(part 1 of 4)
# Autodesk Inventor assembly: 000 Ensamblaje hw_LM - BASIC
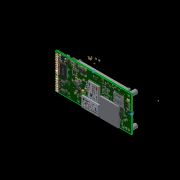
[picture p0: Inventor's stored thumbnail of the model, 180x180]
Saved by Autodesk Inventor 2018.3 (Build 223284000, 284)
## iProperties
Created: 2025-09-15
Part Number: 000 Ensamblaje hw_LM - BASIC
Document SubType Name: Assembly
Designer: mbs18
Mass: 915.711 g
Surface Area: 945.94 cm^2
Volume: 71.5532 cm^3
Density: 12.7976 g/cm^3
Author: mbs18
## Documents named in this file (64)
- C:\Users\mbs18.Embention\Git\LM\items\3d_LM\hw_LM\3d\000 Ensamblaje hw_LM - BASIC.iam
- C:\Users\mbs18.Embention\Git\LM\items\3d_LM\hw_LM\3d\hw_LM - PCB.ipt
- C:\Users\mbs18.Embention\Git\LM\items\_accesories\Componentes PCB\Conectores\3d_Molex\3d\47219-2001\47219-2001.ipt
- C:\Users\mbs18.Embention\Git\LM\items\_accesories\Componentes PCB\Magnetometro\3d_PNI Corp\3d\RM3100\Sen-XY-f.ipt
- C:\Users\mbs18.Embention\Git\LM\items\_accesories\Componentes PCB\Magnetometro\3d_PNI Corp\3d\RM3100\Sen-Z-f.ipt
- C:\Users\mbs18.Embention\Git\LM\items\_accesories\Componentes PCB\Conectores\3d_Samtec\3d\CLP-104-02-F-D-BE-TR.ipt
- C:\Users\mbs18.Embention\Git\LM\items\_accesories\Componentes PCB\Magnetometro\3d_PNI Corp\3d\RM3100\MAGI2C.ipt
- C:\Users\mbs18.Embention\Git\LM\items\_accesories\Componentes PCB\Resistencias\3d_Genérico\R0805.ipt
- C:\Users\mbs18.Embention\Git\LM\items\_accesories\Componentes PCB\Resistencias\3d_Mouser Electronics\3d\ERJ-U02F1601X\RES-1.6K_1%_0402.iam
- C:\Users\mbs18.Embention\Git\LM\items\_accesories\Componentes PCB\Conversores\CC-CC\3d_MuRata\3d\3d_MGJ1D121505MPC-R7\UND_0201CR___ _________.ipt
- C:\Users\mbs18.Embention\Git\LM\items\_accesories\Componentes PCB\Led\3d_ROHM EXCELED\3d\SML-D12V8WT86C.ipt
- C:\Users\mbs18.Embention\Git\LM\items\_accesories\Componentes PCB\Ferrita\3d_Murata Electronics\3d\BLM21PG220SN1D\BLM21PG220SN1D.ipt
- C:\Users\mbs18.Embention\Git\LM\items\_accesories\Componentes PCB\Capacitadores\3d_Kemet\3d\C1206C152KGRACAUTO.ipt
- C:\Users\mbs18.Embention\Git\LM\items\_accesories\Componentes PCB\Diodos\3d_Littlefuse\3d\AQ24CANFD-02HTG\AQ24CANFD-02HTG.ipt
- C:\Users\mbs18.Embention\Git\LM\items\_accesories\Componentes PCB\Jetson Orin Nano\Nvidia\Jetson_Orin_Nano_DevKit_3D_STEP_Model\095-0180-000-TS1_ASM.iam
- C:\Users\mbs18.Embention\Git\LM\items\_accesories\Componentes PCB\Microcontroladores\S32E288ABCAAMJGT.ipt
- C:\Users\mbs18.Embention\Git\LM\items\_accesories\Componentes PCB\Transceptor\3d_Texas Instrument\3d\DP83867ERGZT\DP83867ERGZT.iam
- C:\Users\mbs18.Embention\Git\LM\items\_accesories\Componentes PCB\CAN\3d\3d_Texas_Instruments\TCAN1462VDRBRQ1\TCAN1462VDRBRQ1.iam
- C:\Users\mbs18.Embention\Git\LM\items\_accesories\Componentes PCB\Diodos\3d_Bourns\3d\SMA6J64CA\SMA6J64CA.ipt
- C:\Users\mbs18.Embention\Git\LM\items\_accesories\Componentes PCB\Condensadores\3d_KEMET\3d\C1210C472KGRACAUTO\C1210C472KGRACAUTO.ipt
- C:\Users\mbs18.Embention\Git\LM\items\_accesories\Componentes PCB\Condensadores\3d_KEMET\3d\C0603C103K1RECAUTO\C0603C103K1RECAUTO.iam
- C:\Users\mbs18.Embention\Git\LM\items\_accesories\Componentes PCB\DC-DC\3d_Texas Instruments\3d\LM5146QRGYRQ1\LM5146QRGYRQ1.iam
- C:\Users\mbs18.Embention\Git\LM\items\_accesories\Componentes PCB\Bobinas\3d_COILCRAFT\3d\1812CAN-113NRC\1812CAN-113NRC.iam
- C:\Users\mbs18.Embention\Git\LM\items\_accesories\Componentes PCB\CAN\3d\Analog Devices\LTC2875MPDD#PBF.ipt
- C:\Users\mbs18.Embention\Git\LM\items\_accesories\Componentes PCB\Transceptor\3d_Texas Instrument\3d\UQFN-16.ipt
- C:\Users\mbs18.Embention\Git\LM\items\_accesories\Componentes PCB\Oscilador\3d_ECS_International\ECS-400-8-33Q-ADS-TR.ipt
- C:\Users\mbs18.Embention\Git\LM\items\_accesories\Componentes PCB\DC-DC\3d_Texas Instruments\3d\TPS3897ADRYT.ipt
- C:\Users\mbs18.Embention\Git\LM\items\_accesories\Componentes PCB\ESD Protection\3d_Nexperia\3d\PESD2CANFD27V-UX\PESD2CANFD27V-UX.iam
- C:\Users\mbs18.Embention\Git\LM\items\_accesories\Componentes PCB\Diodos\3d_Diodes Incorporated\3d\DMN2710UTQ-7\DMN2710UTQ-7.ipt
- C:\Users\mbs18.Embention\Git\LM\items\_accesories\Componentes PCB\Multiplexor\3d_TI\3d\SN74LVC1G08QDCKRQ1\SN74LVC1G08QDCKRQ1.ipt
- C:\Users\mbs18.Embention\Git\LM\items\_accesories\Componentes PCB\Bobinas\3d_COILCRAFT\3d\XAL7030-472MEC\XAL7030-472MEC.iam
- C:\Users\mbs18.Embention\Git\LM\items\_accesories\Componentes PCB\Inductor\3d_TDK\3d\XAL4020-601MEC\XAL4020-601MEC.ipt
- C:\Users\mbs18.Embention\Git\LM\items\_accesories\Componentes PCB\Diodos\3d_Texas Instrument\3d\TPD4E05U06QDQARQ1.ipt
- C:\Users\mbs18.Embention\Git\LM\items\_accesories\Componentes PCB\Diodos\3d_Littlefuse\3d\AQ05C-01FTG\AQ05C-01FTG.ipt
- C:\Users\mbs18.Embention\Git\LM\items\_accesories\Componentes PCB\GSM\3d_U-blox\3d\Sara\SARA.iam
- C:\Users\mbs18.Embention\Git\LM\items\_accesories\Componentes PCB\GPS - GNSS\3d_U-blox\3d\ZED F9P\u-blox ZED-F9P.ipt
- C:\Users\mbs18.Embention\Git\LM\items\_accesories\Ordenadores y Tablets\3d_NVIDIA\3d\Orin nano\Heatsink\ATS-NVP-3281-C2-R0.ipt
- C:\Users\mbs18.Embention\Git\LM\items\_accesories\AUAV-L10D-M25125-RR-N.ipt
- C:\Users\mbs18.Embention\Git\LM\items\_accesories\Componentes PCB\DC-DC\3d_Linear Technology\3d\LTC7103MPUHE#PBF.ipt
- C:\Users\mbs18.Embention\Git\LM\items\_accesories\Componentes PCB\Active-low load\3d_Texas_Instruments\TPS22910AYZVR\Body.ipt
- C:\Users\mbs18.Embention\Git\LM\items\3d_LM\3d\3d_LM - chapa.ipt
- C:\Users\mbs18.Embention\Git\LM\items\_accesories\Cables y conectores\3d_Hirose Electric Co Ltd\3d\UFL\U.FL-R-SMT-1.ipt
- C:\Users\mbs18.Embention\Git\LM\items\_accesories\Componentes PCB\Transformadores de señal\3d_Wurth Electroniks\3d\749020112B\749020112B.ipt
- C:\Users\mbs18.Embention\Git\LM\items\_accesories\Componentes PCB\Mosfet\3d_Vishay\3d\SQJ402EP-T1_GE3\SQJ402EP-T1_GE3.ipt
- C:\Users\mbs18.Embention\Git\LM\items\_accesories\Componentes PCB\Condensadores\3d_KEMET\3d\T495B107M006ATE700\T495B107M006ATE700\T495B107M006ATE700.ipt
- C:\Users\mbs18.Embention\Git\LM\items\_accesories\Componentes PCB\Reguladores\3d_Texas Instruments\3d\TPS7A5301QRGRRQ1\TPS7A5301QRGRRQ1.iam
- C:\Users\mbs18.Embention\Git\LM\items\_accesories\Componentes PCB\SIM\3d_EMNIFY\3d\ESIM 638037665970.ipt
- C:\Users\mbs18.Embention\Git\LM\items\_accesories\Componentes PCB\Resistencias\3d_Kemet\3d\C0805X104K5RAC3316.ipt
- C:\Users\mbs18.Embention\Git\LM\items\_accesories\Componentes PCB\Reguladores\3d_Texas Instruments\3d\TPS57112CQRTERQ1\TPS57112CQRTERQ1.iam
- C:\Users\mbs18.Embention\Git\LM\items\_accesories\Componentes PCB\Oscilador\3d_ECS_International\ECS-2520MVQ-250-CN-TR\ECS-2520MVQ-250-CN-TR.ipt
- C:\Users\mbs18.Embention\Git\LM\items\_accesories\Cables y conectores\3d_Te Connectivity\3d\2309411-1\2309409-2-1.ipt
- C:\Users\mbs18.Embention\Git\LM\items\_accesories\Componentes PCB\Rectificadores\3d_Vishay\3d\AU3PM-M3_86A.ipt
- C:\Users\mbs18.Embention\Git\LM\items\_accesories\Componentes PCB\Inductor\3d_Vishay\IHLP2020CZER2R2MA1\IHLP2020CZER220M11.ipt
- C:\Users\mbs18.Embention\Git\LM\items\_accesories\Componentes PCB\Schottky Diodes\3d_STMicroelectronics\3d\STPST8H100SFY.ipt
- C:\Users\mbs18.Embention\Git\LM\items\_accesories\Componentes PCB\Reguladores\3d_Texas Instruments\3d\TPS74501PQWDRBRQ1\TPS74501PQWDRBRQ1.iam
- C:\Users\mbs18.Embention\Git\LM\items\_accesories\Componentes PCB\IMU\3d_Bosch\3d\BMI088.ipt
- C:\Users\mbs18.Embention\Git\LM\items\_accesories\Componentes PCB\Jetson Orin Nano\Nvidia\Jetson_Orin_NX_Orin_Nano_Module_3D_STEP_Model_20230310\P3767-pcba-envelop_20230310-modificada.ipt
- C:\Users\mbs18.Embention\Git\LM\items\_accesories\Separadores y torretas\Internal\Steel\3d_Wurth\3d\9774027151R (M2,5x2,7).ipt
- C:\Users\mbs18.Embention\Git\LM\items\_accesories\Separadores y torretas\Internal\Steel\3d_Wurth\3d\9774090360R (M3x9).ipt
- C:\Users\mbs18.Embention\Git\LM\items\_accesories\Componentes PCB\Mosfet\3d_Onsemi\SOT-363-6_2P2X1P35_ONS.ipt
- C:\Users\mbs18.Embention\Git\LM\items\_accesories\Componentes PCB\IMU\3d_TDK\IAM-20680HT.ipt
- C:\Users\mbs18.Embention\Git\LM\items\_accesories\Componentes PCB\IMU\3d_STM\ASM330LHBG1TR.ipt
- C:\Users\mbs18.Embention\Git\LM\items\_accesories\Componentes PCB\DC-DC\3d_Murata\MGJ1D151505MPC\UND_0201CR___ _________.ipt
- C:\Users\mbs18.Embention\Git\LM\items\_accesories\Ordenadores y Tablets\3d_NVIDIA\3d\Orin nano\Cooling Kit for NVIDIA Jetson Xavier NX - screws-harness.ipt
## Components (704 placed, 62 different names)
1. 2309409-2-1:1 — Mate:230, Mate:231, Mate:232, Angle:184
2. hw_LM - PCB:1 — Mate:1, Flush:1, Flush:2, Mate:33, Mate:35, Mate:60, Mate:72, Mate:84, Mate:94, Mate:95, Mate:107, Mate:108, Mate:109, Mate:110, Mate:112, Mate:113, Mate:114, Mate:115, Mate:116, Mate:117, Mate:118, Mate:123, Mate:124, Mate:131, Mate:132, Angle:59, Mate:134, Angle:62, Mate:135, Angle:64, Mate:136, Mate:139, Mate:153, Mate:154, Mate:155, Angle:91, Mate:187, Mate:188, Mate:194, Angle:142, Mate:199, Angle:149, Mate:200, Mate:203, Mate:210, Mate:213, Mate:216, Mate:219, Mate:220, Mate:222, Mate:224, Mate:225, Mate:226, Mate:227, Flush:634, Mate:229, Mate:230, Mate:231, Mate:232, Mate:237, Angle:169, Mate:238, Mate:239, Mate:240, Mate:241, Mate:242, Mate:243, Mate:245, Mate:246, Mate:247, Mate:248, Angle:176, Mate:249, Angle:177, Angle:178, Mate:250, Mate:251, Angle:179, Mate:252, Mate:256, Angle:181, Angle:182, Mate:257, Mate:258, Angle:183, Mate:259, Mate:267, Mate:268, Mate:269, Mate:270, Angle:185, Mate:271, Mate:272, Mate:273, Mate:274, Angle:189, Mate:275, Mate:276, Angle:193, Mate:277, Mate:278, Angle:194, Mate:279, Mate:280, Mate:281, Mate:282, Angle:195, Angle:198, Mate:285, Mate:286, Mate:287, Mate:290, Mate:291, Mate:292, Mate:293, Mate:294, Mate:295, Mate:296, Mate:297, Mate:298, Angle:306, Mate:299, Mate:300, Mate:301, Mate:302, Mate:303, Mate:304, Mate:305, Mate:306, Mate:307
3. 095-0180-000-TS1_ASM:1 [sub-assembly]
4. 47219-2001:1 — Mate:297
5. Sen-XY-f:1 — Mate:35, Flush:16
6. Sen-Z-f:1 — Mate:33, Angle:142
7. Sen-XY-f:2 — Flush:16
8. MAGI2C:1 — Mate:60
9. UND_0201CR___ _________:2
10. BLM21PG220SN1D:4 — Mate:247, Angle:189
11. C1206C152KGRACAUTO:3 — Flush:677
12. S32E288ABCAAMJGT:1 — Mate:94
13. DP83867ERGZT:1 [sub-assembly] — Mate:95
14. SML-D12V8WT86C:2 — Mate:107, Flush:202, Flush:611
15. SML-D12V8WT86C:3 — Mate:108
16. SML-D12V8WT86C:4 — Mate:109
17. SML-D12V8WT86C:5 — Mate:110
18. SML-D12V8WT86C:6 — Flush:202
19. SMA6J64CA:1 — Mate:116, Angle:63
20. SMA6J64CA:2 — Mate:117
21. C1210C472KGRACAUTO:1 — Mate:118
22. 1812CAN-113NRC:1 [sub-assembly] — Mate:123, Flush:635
23. TCAN1462VDRBRQ1:5 [sub-assembly] — Mate:124, Flush:625
24. C1210C472KGRACAUTO:11 — Flush:228, Flush:230, Flush:232
25. C1210C472KGRACAUTO:12 — Flush:228, Flush:230, Flush:232, Flush:629
26. LTC2875MPDD#PBF:1 — Mate:131, Flush:331
27. UQFN-16:1 — Mate:132, Angle:59
28. LTC2875MPDD#PBF:2 — Flush:331
29. TPS3897ADRYT:1 — Mate:134
30. PESD2CANFD27V-UX:1 [sub-assembly] — Angle:62, Mate:135, Angle:63, Flush:650
31. DMN2710UTQ-7:1 — Angle:64, Mate:136
32. C0603C103K1RECAUTO:13 [sub-assembly] — Flush:662
33. C0603C103K1RECAUTO:14 [sub-assembly] — Flush:336, Angle:175, Flush:1144
34. C0603C103K1RECAUTO:15 [sub-assembly] — Flush:336, Flush:653, Flush:660
35. DMN2710UTQ-7:7 — Flush:423, Flush:603
36. DMN2710UTQ-7:8 — Flush:423
37. C0603C103K1RECAUTO:18 [sub-assembly] — Mate:304
38. C0603C103K1RECAUTO:19 [sub-assembly] — Flush:1147
39. C0603C103K1RECAUTO:21 [sub-assembly] — Flush:1148
40. XAL7030-472MEC:2 [sub-assembly]
41. C1206C152KGRACAUTO:8
42. R0805:5
43. XAL4020-601MEC:3 — Mate:188, Flush:627
44. TPD4E05U06QDQARQ1:1 — Mate:153, Flush:447
45. TPD4E05U06QDQARQ1:2 — Flush:448
46. TPD4E05U06QDQARQ1:3 — Flush:447, Flush:448, Flush:614
47. SARA:1 [sub-assembly] — Mate:194, Angle:200
48. SN74LVC1G08QDCKRQ1:2 — Angle:178
49. DMN2710UTQ-7:10 — Flush:603
50. LTC7103MPUHE#PBF:1 — Mate:187
51. SML-D12V8WT86C:7 — Flush:611
52. 749020112B:1 — Mate:199, Angle:149
53. 749020112B:2 — Mate:200
54. AQ05C-01FTG:2
55. AQ24CANFD-02HTG:8 — Mate:203, Angle:198, Angle:201
56. TPD4E05U06QDQARQ1:4 — Flush:614, Flush:615
57. TPD4E05U06QDQARQ1:5 — Flush:615
58. SQJ402EP-T1_GE3:1 — Mate:210, Mate:238
59. TPD4E05U06QDQARQ1:6 — Mate:213
60. T495B107M006ATE700:3 — Mate:216, Flush:652, Angle:195
61. TCAN1462VDRBRQ1:6 [sub-assembly] — Flush:625
62. XAL4020-601MEC:6 — Flush:627
63. SQJ402EP-T1_GE3:2 — Mate:219, Mate:220, Angle:176
64. C1210C472KGRACAUTO:19 — Mate:222
65. C1210C472KGRACAUTO:20 — Flush:629
66. C0805X104K5RAC3316:3 — Flush:631, Angle:197
67. C0805X104K5RAC3316:4 — Flush:631
68. TPS57112CQRTERQ1:1 [sub-assembly] — Mate:224
69. C0805X104K5RAC3316:5 — Flush:632
70. C0805X104K5RAC3316:6 — Flush:632
71. AQ05C-01FTG:3 — Mate:225
72. ECS-2520MVQ-250-CN-TR:1 — Mate:226
73. TCAN1462VDRBRQ1:7 [sub-assembly] — Mate:227
74. AUAV-L10D-M25125-RR-N:2 — Mate:229
75. AU3PM-M3_86A:1 — Mate:237, Angle:169
76. TPS7A5301QRGRRQ1:2 [sub-assembly] — Mate:239, Angle:304
77. U.FL-R-SMT-1:1 — Mate:241
78. U.FL-R-SMT-1:2 — Mate:240, Angle:197
79. u-blox ZED-F9P:1 — Mate:242, Angle:186
80. 1812CAN-113NRC:3 [sub-assembly] — Flush:635
81. IHLP2020CZER220M11:1 — Mate:243
82. R0805:11 — Mate:245
83. CLP-104-02-F-D-BE-TR:1 — Mate:246
84. LM5146QRGYRQ1:1 [sub-assembly] — Mate:248, Angle:175
85. STPST8H100SFY:1 — Mate:249, Angle:177
86. R0805:12 — Flush:638, Angle:191
87. R0805:13 — Flush:638, Angle:191
88. ESIM 638037665970:1 — Mate:250
89. ECS-400-8-33Q-ADS-TR:1 — Mate:251, Angle:179
90. TPS74501PQWDRBRQ1:1 [sub-assembly] — Mate:252, Flush:640
91. TPS74501PQWDRBRQ1:2 [sub-assembly] — Flush:640
92. SN74LVC1G08QDCKRQ1:3 — Mate:256, Angle:181
93. DMN2710UTQ-7:11 — Angle:182, Mate:257, Mate:258, Flush:647
94. DMN2710UTQ-7:12 — Flush:646, Flush:647, Angle:184, Flush:656
95. DMN2710UTQ-7:13 — Flush:646, Angle:183
96. Body:1 — Mate:259, Flush:648
97. Body:2 — Flush:648
98. PESD2CANFD27V-UX:4 [sub-assembly] — Flush:650
99. 9774027151R (M2,5x2,7):1 — Mate:262, Mate:263
100. 9774027151R (M2,5x2,7):2 — Mate:260, Mate:261
101. 9774090360R (M3x9):1 — Mate:267, Mate:268, Flush:651
102. 9774090360R (M3x9):2 — Flush:651, Mate:269
103. 9774090360R (M3x9):3 — Mate:270, Mate:272
104. T495B107M006ATE700:5 — Flush:652
105. SOT-363-6_2P2X1P35_ONS:1 — Angle:185, Mate:271, Angle:186
106. C1210C472KGRACAUTO:21 — Mate:273, Angle:188
107. C1210C472KGRACAUTO:22 — Mate:274, Angle:188
108. T495B107M006ATE700:6 — Mate:275
109. BMI088:1 — Mate:276, Angle:193
110. C0603C103K1RECAUTO:29 [sub-assembly] — Flush:653, Flush:659
111. C1206C152KGRACAUTO:9 — Mate:277, Flush:1146, Flush:1149
112. Body:4 — Mate:278
113. DMN2710UTQ-7:14 — Flush:656, Angle:194
114. AQ05C-01FTG:4 — Mate:279, Mate:280
115. C0603C103K1RECAUTO:33 [sub-assembly] — Flush:659
116. IAM-20680HT:1 — Mate:281, Flush:671
117. ASM330LHBG1TR:1 — Mate:282
118. C0603C103K1RECAUTO:34 [sub-assembly] — Flush:660, Flush:661, Flush:663
119. C0603C103K1RECAUTO:35 [sub-assembly] — Flush:661
120. C0603C103K1RECAUTO:36 [sub-assembly] — Flush:662, Flush:663
121. IAM-20680HT:2 — Flush:671
122. C1206C152KGRACAUTO:10 — Flush:677
123. R0805:14 — Mate:285
124. C0603C103K1RECAUTO:42 [sub-assembly] — Mate:286, Flush:678
125. C0603C103K1RECAUTO:44 [sub-assembly] — Flush:678
126. C0603C103K1RECAUTO:50 [sub-assembly] — Angle:305, Mate:299, Flush:1147, Flush:1148
127. C0603C103K1RECAUTO:52 [sub-assembly] — Angle:304, Angle:305, Mate:298, Flush:1145
128. C0603C103K1RECAUTO:53 [sub-assembly]
129. C0603C103K1RECAUTO:54 [sub-assembly] — Flush:1152, Flush:1153, Flush:1155
130. C0603C103K1RECAUTO:55 [sub-assembly] — Flush:1153, Flush:1155, Flush:1156
131. C0603C103K1RECAUTO:56 [sub-assembly] — Flush:1158
132. C0603C103K1RECAUTO:57 [sub-assembly] — Flush:1152, Flush:1154
133. C0603C103K1RECAUTO:58 [sub-assembly]
134. C0603C103K1RECAUTO:59 [sub-assembly] — Flush:1156
135. C0603C103K1RECAUTO:60 [sub-assembly] — Mate:305, Flush:1158
136. C0603C103K1RECAUTO:61 [sub-assembly] — Mate:303
137. C0603C103K1RECAUTO:62 [sub-assembly] — Flush:1145
138. C0603C103K1RECAUTO:63 [sub-assembly] — Mate:307
139. C0603C103K1RECAUTO:64 [sub-assembly] — Flush:1157
140. C0603C103K1RECAUTO:65 [sub-assembly] — Mate:292
141. C0603C103K1RECAUTO:66 [sub-assembly] — Mate:291
142. C0603C103K1RECAUTO:67 [sub-assembly] — Mate:294
143. C0603C103K1RECAUTO:68 [sub-assembly] — Mate:290
144. C0603C103K1RECAUTO:69 [sub-assembly] — Mate:301
145. C0603C103K1RECAUTO:70 [sub-assembly] — Mate:302
146. C0603C103K1RECAUTO:71 [sub-assembly] — Mate:293
147. C0603C103K1RECAUTO:72 [sub-assembly] — Mate:306
148. C0603C103K1RECAUTO:73 [sub-assembly] — Mate:300, Flush:1150, Flush:1154, Flush:1157
149. C0603C103K1RECAUTO:74 [sub-assembly] — Mate:296, Flush:1144
150. C0603C103K1RECAUTO:75 [sub-assembly] — Flush:1151
151. C0603C103K1RECAUTO:76 [sub-assembly] — Flush:1150, Flush:1151
152. C0603C103K1RECAUTO:77 [sub-assembly] — Mate:295
153. C1206C152KGRACAUTO:11 — Flush:1146, Angle:306
154. C1206C152KGRACAUTO:12 — Flush:1149
155. Cooling Kit for NVIDIA Jetson Xavier NX - screws-harness:1 — Flush:1143, Mate:288, Mate:289
156. ATS-NVP-3281-C2-R0:1 — Mate:171
157. 3d_LM - chapa:1 — Mate:266, Mate:283, Mate:284
158. P3767-pcba-envelop_20230310-modificada:1 — Mate:154, Mate:155, Mate:171, Flush:634, Mate:260, Mate:261, Mate:262, Mate:263, Mate:266, Mate:283, Mate:284, Flush:1143, Mate:288, Mate:289
159. RES-1.6K_1%_0402:9 [sub-assembly] — Flush:59
160. RES-1.6K_1%_0402:332 [sub-assembly] — Flush:1070, Flush:1078
161. RES-1.6K_1%_0402:263 [sub-assembly] — Angle:95, Flush:517, Flush:535
162. RES-1.6K_1%_0402:1 [sub-assembly] — Mate:72
163. RES-1.6K_1%_0402:8 [sub-assembly] — Flush:59
164. RES-1.6K_1%_0402:10 [sub-assembly]
165. RES-1.6K_1%_0402:13 [sub-assembly] — Flush:66
166. RES-1.6K_1%_0402:14 [sub-assembly] — Flush:64, Flush:65
167. RES-1.6K_1%_0402:15 [sub-assembly] — Flush:65, Flush:66
168. RES-1.6K_1%_0402:16 [sub-assembly] — Flush:64, Flush:73, Flush:118
169. RES-1.6K_1%_0402:18 [sub-assembly] — Flush:73
170. RES-1.6K_1%_0402:20 [sub-assembly]
171. RES-1.6K_1%_0402:21 [sub-assembly]
172. RES-1.6K_1%_0402:22 [sub-assembly] — Flush:85, Flush:86
173. RES-1.6K_1%_0402:25 [sub-assembly]
174. RES-1.6K_1%_0402:27 [sub-assembly] — Flush:85
175. RES-1.6K_1%_0402:28 [sub-assembly]
176. RES-1.6K_1%_0402:29 [sub-assembly] — Flush:86
177. RES-1.6K_1%_0402:31 [sub-assembly]
178. RES-1.6K_1%_0402:34 [sub-assembly]
179. RES-1.6K_1%_0402:35 [sub-assembly] — Flush:676
180. RES-1.6K_1%_0402:38 [sub-assembly]
181. RES-1.6K_1%_0402:40 [sub-assembly] — Flush:118
182. RES-1.6K_1%_0402:42 [sub-assembly]
183. RES-1.6K_1%_0402:44 [sub-assembly] — Flush:138
184. RES-1.6K_1%_0402:45 [sub-assembly]
185. RES-1.6K_1%_0402:48 [sub-assembly]
186. RES-1.6K_1%_0402:49 [sub-assembly]
187. RES-1.6K_1%_0402:50 [sub-assembly] — Flush:153
188. RES-1.6K_1%_0402:51 [sub-assembly] — Flush:153
189. RES-1.6K_1%_0402:53 [sub-assembly]
190. RES-1.6K_1%_0402:56 [sub-assembly] — Flush:138, Mate:84, Flush:146, Flush:151
191. RES-1.6K_1%_0402:58 [sub-assembly] — Flush:146
192. RES-1.6K_1%_0402:59 [sub-assembly] — Flush:151
193. RES-1.6K_1%_0402:60 [sub-assembly] — Flush:159
194. RES-1.6K_1%_0402:61 [sub-assembly] — Flush:160
195. RES-1.6K_1%_0402:62 [sub-assembly] — Flush:164, Flush:168
196. RES-1.6K_1%_0402:63 [sub-assembly] — Flush:159, Flush:160
197. RES-1.6K_1%_0402:64 [sub-assembly]
198. RES-1.6K_1%_0402:65 [sub-assembly] — Flush:164
199. RES-1.6K_1%_0402:66 [sub-assembly] — Flush:183
200. RES-1.6K_1%_0402:67 [sub-assembly] — Flush:182
201. RES-1.6K_1%_0402:69 [sub-assembly] — Flush:168
202. RES-1.6K_1%_0402:71 [sub-assembly]
203. RES-1.6K_1%_0402:72 [sub-assembly] — Flush:174
204. RES-1.6K_1%_0402:73 [sub-assembly]
205. RES-1.6K_1%_0402:75 [sub-assembly] — Flush:174
206. RES-1.6K_1%_0402:76 [sub-assembly] — Flush:183
207. RES-1.6K_1%_0402:77 [sub-assembly]
208. RES-1.6K_1%_0402:78 [sub-assembly] — Flush:186
209. RES-1.6K_1%_0402:79 [sub-assembly] — Flush:182
210. RES-1.6K_1%_0402:80 [sub-assembly] — Flush:186
211. RES-1.6K_1%_0402:81 [sub-assembly]
212. RES-1.6K_1%_0402:84 [sub-assembly] — Flush:192, Angle:199
213. RES-1.6K_1%_0402:85 [sub-assembly] — Flush:192, Flush:194
214. RES-1.6K_1%_0402:86 [sub-assembly] — Flush:194
215. RES-1.6K_1%_0402:88 [sub-assembly]
216. RES-1.6K_1%_0402:89 [sub-assembly] — Mate:115, Flush:204, Flush:205
217. RES-1.6K_1%_0402:90 [sub-assembly] — Mate:114, Flush:205, Flush:206
218. RES-1.6K_1%_0402:91 [sub-assembly] — Mate:113, Flush:206, Flush:207
219. RES-1.6K_1%_0402:92 [sub-assembly] — Mate:112, Flush:207
220. RES-1.6K_1%_0402:94 [sub-assembly] — Flush:204
221. RES-1.6K_1%_0402:97 [sub-assembly] — Mate:139, Flush:451, Flush:467, Flush:479, Flush:492, Flush:518
222. RES-1.6K_1%_0402:101 [sub-assembly]
223. RES-1.6K_1%_0402:104 [sub-assembly] — Flush:251
224. RES-1.6K_1%_0402:105 [sub-assembly] — Flush:252, Flush:261, Flush:278
225. RES-1.6K_1%_0402:107 [sub-assembly] — Flush:249, Flush:252
226. RES-1.6K_1%_0402:108 [sub-assembly]
227. RES-1.6K_1%_0402:109 [sub-assembly] — Flush:249, Flush:251
228. RES-1.6K_1%_0402:110 [sub-assembly]
229. RES-1.6K_1%_0402:113 [sub-assembly] — Flush:261, Flush:296, Flush:319
230. RES-1.6K_1%_0402:114 [sub-assembly]
231. RES-1.6K_1%_0402:115 [sub-assembly] — Flush:1142
232. RES-1.6K_1%_0402:117 [sub-assembly] — Flush:295
233. RES-1.6K_1%_0402:118 [sub-assembly]
234. RES-1.6K_1%_0402:120 [sub-assembly] — Flush:278
235. RES-1.6K_1%_0402:121 [sub-assembly]
236. RES-1.6K_1%_0402:123 [sub-assembly]
237. RES-1.6K_1%_0402:124 [sub-assembly]
238. RES-1.6K_1%_0402:128 [sub-assembly]
239. RES-1.6K_1%_0402:129 [sub-assembly]
240. RES-1.6K_1%_0402:130 [sub-assembly]
241. RES-1.6K_1%_0402:131 [sub-assembly]
242. RES-1.6K_1%_0402:132 [sub-assembly]
243. RES-1.6K_1%_0402:133 [sub-assembly]
244. RES-1.6K_1%_0402:134 [sub-assembly] — Flush:294
245. RES-1.6K_1%_0402:135 [sub-assembly]
246. RES-1.6K_1%_0402:136 [sub-assembly]
247. RES-1.6K_1%_0402:137 [sub-assembly] — Flush:296
248. RES-1.6K_1%_0402:138 [sub-assembly]
249. RES-1.6K_1%_0402:139 [sub-assembly] — Flush:294, Flush:295
250. RES-1.6K_1%_0402:140 [sub-assembly]
251. RES-1.6K_1%_0402:141 [sub-assembly]
252. RES-1.6K_1%_0402:142 [sub-assembly]
253. RES-1.6K_1%_0402:143 [sub-assembly] — Flush:327
254. RES-1.6K_1%_0402:144 [sub-assembly] — Flush:324
255. RES-1.6K_1%_0402:145 [sub-assembly] — Flush:317, Flush:328
256. RES-1.6K_1%_0402:146 [sub-assembly] — Flush:326, Flush:346
257. RES-1.6K_1%_0402:147 [sub-assembly] — Flush:318
258. RES-1.6K_1%_0402:148 [sub-assembly]
259. RES-1.6K_1%_0402:149 [sub-assembly]
260. RES-1.6K_1%_0402:150 [sub-assembly] — Flush:319
261. RES-1.6K_1%_0402:151 [sub-assembly]
262. RES-1.6K_1%_0402:155 [sub-assembly] — Flush:318
263. RES-1.6K_1%_0402:156 [sub-assembly]
264. RES-1.6K_1%_0402:157 [sub-assembly] — Flush:317
265. RES-1.6K_1%_0402:158 [sub-assembly]
266. RES-1.6K_1%_0402:159 [sub-assembly]
267. RES-1.6K_1%_0402:160 [sub-assembly] — Flush:326
268. RES-1.6K_1%_0402:161 [sub-assembly] — Flush:324, Flush:325, Flush:328
269. RES-1.6K_1%_0402:162 [sub-assembly] — Flush:325
270. RES-1.6K_1%_0402:164 [sub-assembly] — Flush:327
271. RES-1.6K_1%_0402:166 [sub-assembly]
272. RES-1.6K_1%_0402:168 [sub-assembly] — Flush:346
273. RES-1.6K_1%_0402:170 [sub-assembly] — Flush:382
274. RES-1.6K_1%_0402:178 [sub-assembly]
275. RES-1.6K_1%_0402:179 [sub-assembly]
276. RES-1.6K_1%_0402:180 [sub-assembly]
277. RES-1.6K_1%_0402:181 [sub-assembly]
278. RES-1.6K_1%_0402:182 [sub-assembly]
279. RES-1.6K_1%_0402:183 [sub-assembly] — Flush:382, Flush:383
280. RES-1.6K_1%_0402:184 [sub-assembly]
281. RES-1.6K_1%_0402:185 [sub-assembly] — Flush:384
282. RES-1.6K_1%_0402:186 [sub-assembly] — Angle:73, Angle:74
283. RES-1.6K_1%_0402:187 [sub-assembly] — Flush:386, Angle:74
284. RES-1.6K_1%_0402:188 [sub-assembly] — Flush:387, Angle:75
285. RES-1.6K_1%_0402:189 [sub-assembly] — Flush:388, Angle:71, Angle:72, Angle:75
286. RES-1.6K_1%_0402:190 [sub-assembly] — Angle:70, Angle:71
287. RES-1.6K_1%_0402:191 [sub-assembly] — Angle:69, Angle:70, Flush:398
288. RES-1.6K_1%_0402:192 [sub-assembly] — Angle:69
289. RES-1.6K_1%_0402:193 [sub-assembly] — Angle:72, Angle:73
290. RES-1.6K_1%_0402:194 [sub-assembly]
291. RES-1.6K_1%_0402:195 [sub-assembly] — Angle:199, Angle:200
292. RES-1.6K_1%_0402:196 [sub-assembly]
293. RES-1.6K_1%_0402:197 [sub-assembly] — Flush:386
294. RES-1.6K_1%_0402:198 [sub-assembly] — Flush:383
295. RES-1.6K_1%_0402:200 [sub-assembly] — Flush:384, Flush:388
296. RES-1.6K_1%_0402:201 [sub-assembly] — Flush:387
297. RES-1.6K_1%_0402:202 [sub-assembly] — Flush:398
298. RES-1.6K_1%_0402:203 [sub-assembly]
299. RES-1.6K_1%_0402:207 [sub-assembly]
300. RES-1.6K_1%_0402:208 [sub-assembly]
301. RES-1.6K_1%_0402:209 [sub-assembly]
302. RES-1.6K_1%_0402:210 [sub-assembly]
303. RES-1.6K_1%_0402:211 [sub-assembly]
304. RES-1.6K_1%_0402:212 [sub-assembly]
305. RES-1.6K_1%_0402:213 [sub-assembly]
306. RES-1.6K_1%_0402:214 [sub-assembly]
307. RES-1.6K_1%_0402:215 [sub-assembly] — Flush:417
308. RES-1.6K_1%_0402:216 [sub-assembly]
309. RES-1.6K_1%_0402:218 [sub-assembly]
310. RES-1.6K_1%_0402:221 [sub-assembly] — Flush:417
311. RES-1.6K_1%_0402:222 [sub-assembly]
312. RES-1.6K_1%_0402:224 [sub-assembly] — Flush:452, Flush:466
313. RES-1.6K_1%_0402:225 [sub-assembly] — Flush:453, Flush:454, Flush:595
314. RES-1.6K_1%_0402:226 [sub-assembly] — Flush:450, Flush:451, Flush:452, Flush:453, Flush:467, Flush:476
315. RES-1.6K_1%_0402:227 [sub-assembly] — Flush:450, Flush:454
316. RES-1.6K_1%_0402:228 [sub-assembly] — Flush:465
317. RES-1.6K_1%_0402:231 [sub-assembly]
318. RES-1.6K_1%_0402:232 [sub-assembly] — Flush:477
319. RES-1.6K_1%_0402:233 [sub-assembly] — Flush:465, Flush:669
320. RES-1.6K_1%_0402:234 [sub-assembly] — Flush:479, Flush:480
321. RES-1.6K_1%_0402:235 [sub-assembly] — Flush:466
322. RES-1.6K_1%_0402:236 [sub-assembly] — Flush:478
323. RES-1.6K_1%_0402:237 [sub-assembly] — Flush:477
324. RES-1.6K_1%_0402:238 [sub-assembly]
325. RES-1.6K_1%_0402:239 [sub-assembly] — Flush:476
326. RES-1.6K_1%_0402:240 [sub-assembly] — Flush:480
327. RES-1.6K_1%_0402:241 [sub-assembly] — Flush:478
328. RES-1.6K_1%_0402:242 [sub-assembly]
329. RES-1.6K_1%_0402:243 [sub-assembly] — Flush:1141
330. RES-1.6K_1%_0402:245 [sub-assembly]
331. RES-1.6K_1%_0402:247 [sub-assembly] — Flush:491
332. RES-1.6K_1%_0402:248 [sub-assembly] — Flush:503
333. RES-1.6K_1%_0402:249 [sub-assembly] — Flush:491, Flush:492
334. RES-1.6K_1%_0402:251 [sub-assembly]
335. RES-1.6K_1%_0402:252 [sub-assembly]
336. RES-1.6K_1%_0402:253 [sub-assembly] — Flush:502, Flush:504
337. RES-1.6K_1%_0402:256 [sub-assembly] — Flush:504
338. RES-1.6K_1%_0402:257 [sub-assembly] — Angle:93, Angle:94, Angle:97
339. RES-1.6K_1%_0402:258 [sub-assembly] — Flush:503, Angle:91, Angle:92, Angle:93, Flush:550, Flush:551
340. RES-1.6K_1%_0402:259 [sub-assembly] — Flush:502, Angle:92, Flush:515, Flush:1072, Flush:1073, Flush:1092
341. RES-1.6K_1%_0402:260 [sub-assembly] — Angle:97, Angle:98, Angle:99
342. RES-1.6K_1%_0402:261 [sub-assembly] — Angle:98
343. RES-1.6K_1%_0402:262 [sub-assembly] — Angle:99, Flush:595
344. RES-1.6K_1%_0402:264 [sub-assembly] — Angle:94, Angle:95, Angle:96
345. RES-1.6K_1%_0402:265 [sub-assembly] — Angle:96
346. RES-1.6K_1%_0402:266 [sub-assembly] — Flush:516
347. RES-1.6K_1%_0402:267 [sub-assembly] — Flush:516, Flush:517
348. RES-1.6K_1%_0402:268 [sub-assembly] — Flush:515, Flush:535
349. RES-1.6K_1%_0402:269 [sub-assembly]
350. RES-1.6K_1%_0402:270 [sub-assembly] — Flush:518
351. RES-1.6K_1%_0402:272 [sub-assembly] — Flush:532, Flush:534
352. RES-1.6K_1%_0402:273 [sub-assembly] — Flush:532, Flush:534
353. RES-1.6K_1%_0402:274 [sub-assembly]
354. RES-1.6K_1%_0402:275 [sub-assembly] — Flush:533
355. RES-1.6K_1%_0402:276 [sub-assembly]
356. RES-1.6K_1%_0402:277 [sub-assembly] — Flush:530
357. RES-1.6K_1%_0402:278 [sub-assembly] — Flush:530, Flush:533
358. RES-1.6K_1%_0402:279 [sub-assembly]
359. RES-1.6K_1%_0402:280 [sub-assembly] — Flush:546
360. RES-1.6K_1%_0402:282 [sub-assembly] — Flush:549, Flush:564, Flush:565
361. RES-1.6K_1%_0402:283 [sub-assembly] — Flush:545, Flush:546, Flush:550, Flush:584, Flush:589
362. RES-1.6K_1%_0402:284 [sub-assembly]
363. RES-1.6K_1%_0402:285 [sub-assembly] — Flush:547
364. RES-1.6K_1%_0402:286 [sub-assembly] — Flush:545, Flush:547, Flush:548, Flush:567
365. RES-1.6K_1%_0402:287 [sub-assembly] — Flush:549, Flush:551, Flush:570
366. RES-1.6K_1%_0402:288 [sub-assembly] — Flush:579, Flush:583, Flush:588
367. RES-1.6K_1%_0402:289 [sub-assembly] — Flush:548, Flush:566
368. RES-1.6K_1%_0402:290 [sub-assembly] — Flush:565
369. RES-1.6K_1%_0402:291 [sub-assembly] — Flush:566, Flush:594
370. RES-1.6K_1%_0402:293 [sub-assembly] — Flush:567
371. RES-1.6K_1%_0402:294 [sub-assembly]
372. RES-1.6K_1%_0402:295 [sub-assembly]
373. RES-1.6K_1%_0402:296 [sub-assembly] — Flush:1093
374. RES-1.6K_1%_0402:297 [sub-assembly] — Flush:564
375. RES-1.6K_1%_0402:298 [sub-assembly]
376. RES-1.6K_1%_0402:300 [sub-assembly] — Flush:570
377. RES-1.6K_1%_0402:302 [sub-assembly]
378. RES-1.6K_1%_0402:303 [sub-assembly] — Flush:580
379. RES-1.6K_1%_0402:304 [sub-assembly]
380. RES-1.6K_1%_0402:306 [sub-assembly] — Flush:582, Flush:585, Flush:590
381. RES-1.6K_1%_0402:307 [sub-assembly] — Flush:579
382. RES-1.6K_1%_0402:308 [sub-assembly]
383. RES-1.6K_1%_0402:309 [sub-assembly] — Flush:594
384. RES-1.6K_1%_0402:310 [sub-assembly] — Flush:580
385. RES-1.6K_1%_0402:311 [sub-assembly] — Flush:585, Flush:596
386. RES-1.6K_1%_0402:312 [sub-assembly] — Flush:583, Flush:597
387. RES-1.6K_1%_0402:313 [sub-assembly] — Flush:584
388. RES-1.6K_1%_0402:314 [sub-assembly] — Flush:582
389. RES-1.6K_1%_0402:315 [sub-assembly] — Flush:597
390. RES-1.6K_1%_0402:316 [sub-assembly] — Flush:596
391. RES-1.6K_1%_0402:317 [sub-assembly] — Flush:588
392. RES-1.6K_1%_0402:318 [sub-assembly] — Flush:589
393. RES-1.6K_1%_0402:319 [sub-assembly]
394. RES-1.6K_1%_0402:320 [sub-assembly]
395. RES-1.6K_1%_0402:321 [sub-assembly] — Flush:590
396. RES-1.6K_1%_0402:322 [sub-assembly]
397. RES-1.6K_1%_0402:323 [sub-assembly] — Flush:1141
398. RES-1.6K_1%_0402:324 [sub-assembly]
399. RES-1.6K_1%_0402:325 [sub-assembly]
400. RES-1.6K_1%_0402:326 [sub-assembly]
401. RES-1.6K_1%_0402:327 [sub-assembly] — Flush:669, Flush:670
402. RES-1.6K_1%_0402:328 [sub-assembly] — Flush:670
403. RES-1.6K_1%_0402:329 [sub-assembly] — Flush:674, Flush:676
404. RES-1.6K_1%_0402:330 [sub-assembly] — Flush:675
405. RES-1.6K_1%_0402:331 [sub-assembly] — Flush:674, Flush:675
406. RES-1.6K_1%_0402:333 [sub-assembly] — Flush:1070, Flush:1073, Flush:1075
407. RES-1.6K_1%_0402:334 [sub-assembly] — Flush:1071
408. RES-1.6K_1%_0402:335 [sub-assembly] — Flush:1071, Flush:1072, Flush:1100
409. RES-1.6K_1%_0402:336 [sub-assembly] — Flush:1074
410. RES-1.6K_1%_0402:337 [sub-assembly] — Flush:1075, Flush:1078, Flush:1079
411. RES-1.6K_1%_0402:338 [sub-assembly] — Flush:1077, Flush:1079, Flush:1080
412. RES-1.6K_1%_0402:339 [sub-assembly] — Flush:1074, Flush:1077
413. RES-1.6K_1%_0402:340 [sub-assembly] — Flush:1080, Flush:1082
414. RES-1.6K_1%_0402:341 [sub-assembly] — Flush:1081, Flush:1083, Flush:1091
415. RES-1.6K_1%_0402:342 [sub-assembly] — Flush:1081, Flush:1083
416. RES-1.6K_1%_0402:343 [sub-assembly] — Flush:1082, Flush:1132
417. RES-1.6K_1%_0402:344 [sub-assembly] — Flush:1091
418. RES-1.6K_1%_0402:345 [sub-assembly] — Flush:1090, Flush:1093
419. RES-1.6K_1%_0402:346 [sub-assembly] — Flush:1090, Flush:1116, Flush:1128, Flush:1140
420. RES-1.6K_1%_0402:347 [sub-assembly] — Flush:1092, Flush:1112, Flush:1117
421. RES-1.6K_1%_0402:348 [sub-assembly] — Flush:1099, Flush:1100, Flush:1119
422. RES-1.6K_1%_0402:349 [sub-assembly]
423. RES-1.6K_1%_0402:350 [sub-assembly]
424. RES-1.6K_1%_0402:351 [sub-assembly]
425. RES-1.6K_1%_0402:352 [sub-assembly] — Flush:1099
426. RES-1.6K_1%_0402:353 [sub-assembly]
427. RES-1.6K_1%_0402:354 [sub-assembly] — Flush:1110, Flush:1111
428. RES-1.6K_1%_0402:355 [sub-assembly] — Flush:1109, Flush:1110
429. RES-1.6K_1%_0402:356 [sub-assembly] — Flush:1111
430. RES-1.6K_1%_0402:357 [sub-assembly] — Flush:1109, Flush:1112
431. RES-1.6K_1%_0402:358 [sub-assembly]
432. RES-1.6K_1%_0402:359 [sub-assembly] — Flush:1116
433. RES-1.6K_1%_0402:360 [sub-assembly] — Flush:1118, Flush:1119
434. RES-1.6K_1%_0402:361 [sub-assembly] — Flush:1117, Flush:1118
435. RES-1.6K_1%_0402:362 [sub-assembly] — Flush:1125, Flush:1128
436. RES-1.6K_1%_0402:363 [sub-assembly] — Flush:1126
437. RES-1.6K_1%_0402:364 [sub-assembly] — Flush:1124, Flush:1127
438. RES-1.6K_1%_0402:365 [sub-assembly] — Flush:1127
439. RES-1.6K_1%_0402:366 [sub-assembly] — Flush:1124, Flush:1126
440. RES-1.6K_1%_0402:367 [sub-assembly] — Flush:1125
441. RES-1.6K_1%_0402:368 [sub-assembly] — Flush:1132, Flush:1133, Flush:1134
442. RES-1.6K_1%_0402:369 [sub-assembly] — Flush:1134
443. RES-1.6K_1%_0402:370 [sub-assembly] — Flush:1133
444. RES-1.6K_1%_0402:371 [sub-assembly]
445. RES-1.6K_1%_0402:372 [sub-assembly] — Flush:1140
446. RES-1.6K_1%_0402:373 [sub-assembly] — Flush:1139
447. RES-1.6K_1%_0402:374 [sub-assembly] — Flush:1139
448. RES-1.6K_1%_0402:375 [sub-assembly] — Flush:1142
449. UND_0201CR___ _________:3 — Mate:287, Flush:690, Flush:709
450. UND_0201CR___ _________:4 — Flush:681
451. UND_0201CR___ _________:5 — Flush:679, Flush:683
452. UND_0201CR___ _________:6 — Flush:682, Flush:683, Flush:737, Flush:798
453. UND_0201CR___ _________:7 — Flush:680, Flush:691
454. UND_0201CR___ _________:8 — Flush:679, Flush:680, Flush:681, Flush:692, Flush:706, Flush:772
455. UND_0201CR___ _________:9 — Flush:682, Flush:689, Flush:690
456. UND_0201CR___ _________:10 — Flush:691, Flush:708
457. UND_0201CR___ _________:11 — Flush:689, Flush:692
458. UND_0201CR___ _________:12
459. UND_0201CR___ _________:13
460. UND_0201CR___ _________:14
461. UND_0201CR___ _________:15 — Flush:707
462. UND_0201CR___ _________:16
463. UND_0201CR___ _________:17
464. UND_0201CR___ _________:18 — Flush:707
465. UND_0201CR___ _________:19 — Flush:709
466. UND_0201CR___ _________:20 — Flush:706
467. UND_0201CR___ _________:21
468. UND_0201CR___ _________:22
469. UND_0201CR___ _________:23
470. UND_0201CR___ _________:24
471. UND_0201CR___ _________:25 — Flush:708
472. UND_0201CR___ _________:26
473. UND_0201CR___ _________:27
474. UND_0201CR___ _________:28
475. UND_0201CR___ _________:29
476. UND_0201CR___ _________:30 — Flush:735
477. UND_0201CR___ _________:31
478. UND_0201CR___ _________:32 — Flush:736
479. UND_0201CR___ _________:33 — Flush:737
480. UND_0201CR___ _________:34
481. UND_0201CR___ _________:35 — Flush:734
482. UND_0201CR___ _________:36 — Flush:1130
483. UND_0201CR___ _________:37
484. UND_0201CR___ _________:38
485. UND_0201CR___ _________:39 — Flush:799
486. UND_0201CR___ _________:40 — Flush:735, Flush:772
487. UND_0201CR___ _________:41
488. UND_0201CR___ _________:42
489. UND_0201CR___ _________:43 — Flush:769
490. UND_0201CR___ _________:44 — Flush:768
491. UND_0201CR___ _________:45
492. UND_0201CR___ _________:46
493. UND_0201CR___ _________:47
494. UND_0201CR___ _________:48 — Flush:734
495. UND_0201CR___ _________:49 — Flush:736, Flush:770
496. UND_0201CR___ _________:50 — Flush:794
497. UND_0201CR___ _________:51 — Flush:768
498. UND_0201CR___ _________:52
499. UND_0201CR___ _________:53
500. UND_0201CR___ _________:54
501. UND_0201CR___ _________:55
502. UND_0201CR___ _________:56
503. UND_0201CR___ _________:57 — Flush:770, Flush:797
504. UND_0201CR___ _________:58
505. UND_0201CR___ _________:59
506. UND_0201CR___ _________:60 — Flush:771, Flush:793
507. UND_0201CR___ _________:61
508. UND_0201CR___ _________:62
509. UND_0201CR___ _________:63
510. UND_0201CR___ _________:64 — Flush:792
511. UND_0201CR___ _________:65 — Flush:795
512. UND_0201CR___ _________:66
513. UND_0201CR___ _________:67 — Flush:771, Flush:796, Flush:798
514. UND_0201CR___ _________:68
515. UND_0201CR___ _________:69 — Flush:773
516. UND_0201CR___ _________:70 — Flush:797
517. UND_0201CR___ _________:71
518. UND_0201CR___ _________:72
519. UND_0201CR___ _________:73
520. UND_0201CR___ _________:74
521. UND_0201CR___ _________:75
522. UND_0201CR___ _________:76 — Flush:769
523. UND_0201CR___ _________:77 — Flush:773
524. UND_0201CR___ _________:78
525. UND_0201CR___ _________:79
526. UND_0201CR___ _________:80
527. UND_0201CR___ _________:81 — Flush:819
528. UND_0201CR___ _________:82 — Flush:792
529. UND_0201CR___ _________:83 — Flush:799
530. UND_0201CR___ _________:84 — Flush:794, Flush:823, Flush:860, Flush:889, Flush:1035
531. UND_0201CR___ _________:85
532. UND_0201CR___ _________:86
533. UND_0201CR___ _________:87
534. UND_0201CR___ _________:88 — Flush:793
535. UND_0201CR___ _________:89
536. UND_0201CR___ _________:90 — Flush:795
537. UND_0201CR___ _________:91
538. UND_0201CR___ _________:92 — Flush:796, Flush:818
539. UND_0201CR___ _________:93
540. UND_0201CR___ _________:94
541. UND_0201CR___ _________:95
542. UND_0201CR___ _________:96
543. UND_0201CR___ _________:97
544. UND_0201CR___ _________:98
545. UND_0201CR___ _________:99
546. UND_0201CR___ _________:100
547. UND_0201CR___ _________:101 — Flush:819
548. UND_0201CR___ _________:102
549. UND_0201CR___ _________:103
550. UND_0201CR___ _________:104
551. UND_0201CR___ _________:105
552. UND_0201CR___ _________:106
553. UND_0201CR___ _________:107
554. UND_0201CR___ _________:108 — Flush:818
555. UND_0201CR___ _________:109
556. UND_0201CR___ _________:110
557. UND_0201CR___ _________:111
558. UND_0201CR___ _________:112 — Angle:201, Angle:202, Flush:822, Flush:831
559. UND_0201CR___ _________:113 — Angle:203, Flush:821, Flush:822, Flush:823, Flush:832
560. UND_0201CR___ _________:114 — Angle:202, Angle:203, Flush:821, Flush:830
561. UND_0201CR___ _________:115 — Flush:833
562. UND_0201CR___ _________:116 — Flush:832
563. UND_0201CR___ _________:117 — Flush:830
564. UND_0201CR___ _________:118 — Flush:831, Flush:833
565. UND_0201CR___ _________:119
566. UND_0201CR___ _________:120
567. UND_0201CR___ _________:121
568. UND_0201CR___ _________:122 — Flush:861
569. UND_0201CR___ _________:123
570. UND_0201CR___ _________:124